# Autodesk Inventor assembly: BearingHousing
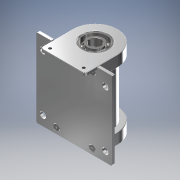
[picture p0: Inventor's stored thumbnail of the model, 180x180]
Saved by Autodesk Inventor 2018 (Build 220112000, 112)
## iProperties
Created: 2018-02-06
Part Number: BearingHousing
Document SubType Name: Weldment
Designer: P136265
Weld Material: Steel, Galvanized
Author: P136265
## Documents named in this file (7)
- C:\Users\P136265\Documents\GitHub\mecanum-cad\BearingHousing.iam
- C:\Users\P136265\Documents\GitHub\mecanum-cad\BearingHousing_Base.ipt
- C:\Users\P136265\Documents\GitHub\mecanum-cad\BearingHousing_Plate.ipt
- C:\Users\P136265\Documents\GitHub\mecanum-cad\BearingHousing_Pipe.ipt
- C:\Users\P136265\Documents\Inventor\Content Center Files\R2018\en-US\SKF B - angular contact\SKF B7204 BE.ipt
- C:\Users\P136265\Documents\GitHub\mecanum-cad\BearingHousing_JackPlate.ipt
- C:\Users\P136265\Documents\Inventor\Content Center Files\R2018\en-US\ASME ANSI B18.3.5M(2)\ASME_ANSI B18.3.5M - M5x12(2).ipt
## Components (10 placed, 6 different names)
1. BearingHousing_Base:1 — Mate:1, Mate:3, Mate:4, Mate:5, Mate:6, Mate:7, Mate:8, Mate:9, Mate:10
2. BearingHousing_Pipe:1 — Mate:2
3. SKF B- Angular contact SKF B7204 BE:1
4. SKF B- Angular contact SKF B7204 BE:2
5. BearingHousing_Plate:1 — Mate:1, Mate:2, Mate:3
6. BearingHousing_JackPlate:1 — Mate:4, Mate:5, Mate:6
7. Broached Hexagon Socket Flat Countersunk Head Cap Screws - Metric M5x12:4 — Mate:7
8. Broached Hexagon Socket Flat Countersunk Head Cap Screws - Metric M5x12:1 — Mate:8
9. Broached Hexagon Socket Flat Countersunk Head Cap Screws - Metric M5x12:2 — Mate:9
10. Broached Hexagon Socket Flat Countersunk Head Cap Screws - Metric M5x12:3 — Mate:10
## Relationships (10: Mate 10)
- Mate:1: BearingHousing_Base:1 ↔ BearingHousing_Plate:1
- Mate:2: BearingHousing_Pipe:1 ↔ BearingHousing_Plate:1
- Mate:3 (1 mm): BearingHousing_Base:1 ↔ BearingHousing_Plate:1
- Mate:4: BearingHousing_Base:1 ↔ BearingHousing_JackPlate:1
- Mate:5: BearingHousing_Base:1 ↔ BearingHousing_JackPlate:1
- Mate:6 (1 mm): BearingHousing_Base:1 ↔ BearingHousing_JackPlate:1
- Mate:7: BearingHousing_Base:1 ↔ Broached Hexagon Socket Flat Countersunk Head Cap Screws - Metric M5x12:4
- Mate:8: BearingHousing_Base:1 ↔ Broached Hexagon Socket Flat Countersunk Head Cap Screws - Metric M5x12:1
- Mate:9: BearingHousing_Base:1 ↔ Broached Hexagon Socket Flat Countersunk Head Cap Screws - Metric M5x12:2
- Mate:10: BearingHousing_Base:1 ↔ Broached Hexagon Socket Flat Countersunk Head Cap Screws - Metric M5x12:3
